# Autodesk Inventor assembly: 276-2181
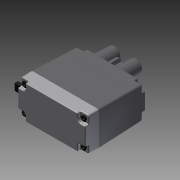
[picture p0: Inventor's stored thumbnail of the model, 180x180]
Saved by Autodesk Inventor 2013 (Build 170138000, 138)
## iProperties
Category: Motors
Company: Autodesk Inc.
Created: 2012-01-28
Part Number: 276-2181
Document SubType Name: Assembly
Designer: Autodesk Inc.
Catalog Web Link: http://www.vexrobotics.com/276-2181.html
Vendor: VEX
Author: Autodesk Inc.
## Documents named in this file (18)
- C:\Data Folder\VEX 2012\VEX KOP Uploads\2013\Imperial\Motion\2-Wire Motor 269.iam
- C:\Data Folder\VEX 2012\VEX KOP Uploads\2013\Imperial\Motion\Components\276-2181-002 Rev1.ipt
- C:\Data Folder\VEX 2012\VEX KOP Uploads\2013\Imperial\Motion\Components\276-2181-006 Rev1.ipt
- C:\Data Folder\VEX 2012\VEX KOP Uploads\2013\Imperial\Motion\Components\276-2181-011 Rev1.ipt
- C:\Data Folder\VEX 2012\VEX KOP Uploads\2013\Imperial\Motion\Components\276-2177-018 Rev1.ipt
- C:\Data Folder\VEX 2012\VEX KOP Uploads\2013\Imperial\Motion\Components\276-2181-004 Rev1.ipt
- C:\Data Folder\VEX 2012\VEX KOP Uploads\2013\Imperial\Motion\Components\276-2181-008 Rev1_276-2181-008g.ipt
- C:\Data Folder\VEX 2012\VEX KOP Uploads\2013\Imperial\Motion\Components\276-2181-007 Rev1.ipt
- C:\Data Folder\VEX 2012\VEX KOP Uploads\2013\Imperial\Motion\Components\276-2181-012 Rev1.ipt
- C:\Data Folder\VEX 2012\VEX KOP Uploads\2013\Imperial\Motion\Components\276-2181-003 Rev1.ipt
- C:\Data Folder\VEX 2012\VEX KOP Uploads\2013\Imperial\Motion\Components\276-2181-001 Rev1.ipt
- C:\Data Folder\VEX 2012\VEX KOP Uploads\2013\Imperial\Motion\Components\QFK-N30QAV-16068.ipt
- C:\Data Folder\VEX 2012\VEX KOP Uploads\2013\Imperial\Motion\Components\ANSI B18.6.3 - 0-80 UNF - 0.1875(14).ipt
- C:\Data Folder\VEX 2012\VEX KOP Uploads\2013\Imperial\Motion\Components\276-2181-010 Rev1.ipt
- C:\Data Folder\VEX 2012\VEX KOP Uploads\2013\Imperial\Motion\Components\276-2181-009 Rev1.ipt
- C:\Data Folder\VEX 2012\VEX KOP Uploads\2013\Imperial\Motion\Components\276-2181-005 Rev1.ipt
- C:\Data Folder\VEX 2012\VEX KOP Uploads\2013\Imperial\Motion\Components\276-2177-019 Rev1.ipt
- C:\Data Folder\VEX 2012\VEX KOP Uploads\2013\Imperial\Motion\Components\ANSI B18.6.3 - 0-80 UNF - 0.5(17).ipt
## Components (29 placed, 17 different names)
1. 276-2181-002 Rev1:1 — Insert:1, Insert:2, Mate:1, Mate:3, Insert:3, Mate:4, Flush:1, Mate:5, Mate:9, Mate:10, Mate:11, Mate:12, Mate:13, Mate:14, Angle:1, Insert:5, Mate:15, Insert:6, Insert:7, Mate:16, Insert:8, Flush:2, Flush:3, Flush:4
2. 276-2181-006 Rev1:1 — Insert:1, Mate:18
3. 276-2181-011 Rev1:1 — Insert:2, Insert:4
4. 276-2177-018 Rev1:1 — Mate:1, Mate:3
5. 276-2181-004 Rev1:1 — Insert:3
6. 276-2181-008 Rev1_276-2181-008g:1 — Insert:4, Insert:9
7. 276-2181-007 Rev1:1 — Mate:4, Flush:1, Mate:7, Mate:8
8. 276-2181-012 Rev1:1 — Mate:5, Angle:1, Mate:19
9. 276-2181-006 Rev1:2 — Mate:7, Mate:8, Mate:17
10. 276-2181-003 Rev1:1 — Mate:9, Mate:10, Mate:14, Insert:10, Insert:11, Insert:16, Insert:17, Insert:18, Insert:19
11. 276-2181-001 Rev1:1 — Mate:11, Mate:12, Mate:13, Insert:12, Insert:13, Insert:14, Insert:15
12. QFK-N30QAV-16068:1 — Insert:5, Mate:15, Mate:19
13. Cross Recessed Binding Head Machine Screw - Type I - Inch 0 - 80 - 3/16:1 — Insert:6
14. Cross Recessed Binding Head Machine Screw - Type I - Inch 0 - 80 - 3/16:2 — Insert:7
15. 276-2181-010 Rev1:1 — Mate:16, Flush:2
16. 276-2181-009 Rev1:1 — Mate:17, Flush:3
17. 276-2181-005 Rev1:1 — Insert:8
18. 276-2181-010 Rev1:2 — Mate:18, Flush:4
19. 276-2181-011 Rev1:2 — Insert:9
20. 276-2177-019 Rev1:1 — Insert:10
21. 276-2177-019 Rev1:2 — Insert:11
22. Cross Recessed Binding Head Machine Screw - Type II - Inch 0 - 80 - 1/2:1 — Insert:12
23. Cross Recessed Binding Head Machine Screw - Type II - Inch 0 - 80 - 1/2:2 — Insert:13
24. Cross Recessed Binding Head Machine Screw - Type II - Inch 0 - 80 - 1/2:4 — Insert:15
25. Cross Recessed Binding Head Machine Screw - Type II - Inch 0 - 80 - 1/2:3 — Insert:14
26. Cross Recessed Binding Head Machine Screw - Type II - Inch 0 - 80 - 1/2:5 — Insert:16
27. Cross Recessed Binding Head Machine Screw - Type II - Inch 0 - 80 - 1/2:6 — Insert:17
28. Cross Recessed Binding Head Machine Screw - Type II - Inch 0 - 80 - 1/2:7 — Insert:18
29. Cross Recessed Binding Head Machine Screw - Type II - Inch 0 - 80 - 1/2:8 — Insert:19
## Relationships (41: Insert 19, Mate 17, Flush 4, Angle 1)
- Insert:1: 276-2181-002 Rev1:1 ↔ 276-2181-006 Rev1:1
- Insert:2: 276-2181-002 Rev1:1 ↔ 276-2181-011 Rev1:1
- Mate:1: 276-2181-002 Rev1:1 ↔ 276-2177-018 Rev1:1
- Mate:3: 276-2181-002 Rev1:1 ↔ 276-2177-018 Rev1:1
- Insert:3: 276-2181-002 Rev1:1 ↔ 276-2181-004 Rev1:1
- Insert:4: 276-2181-011 Rev1:1 ↔ 276-2181-008 Rev1_276-2181-008g:1
- Mate:4: 276-2181-002 Rev1:1 ↔ 276-2181-007 Rev1:1
- Flush:1 (4.191 mm): 276-2181-002 Rev1:1 ↔ 276-2181-007 Rev1:1
- Mate:5: 276-2181-002 Rev1:1 ↔ 276-2181-012 Rev1:1
- Mate:7: 276-2181-007 Rev1:1 ↔ 276-2181-006 Rev1:2
- Mate:8: 276-2181-007 Rev1:1 ↔ 276-2181-006 Rev1:2
- Mate:9: 276-2181-002 Rev1:1 ↔ 276-2181-003 Rev1:1
- Mate:10: 276-2181-002 Rev1:1 ↔ 276-2181-003 Rev1:1
- Mate:11: 276-2181-002 Rev1:1 ↔ 276-2181-001 Rev1:1
- Mate:12: 276-2181-002 Rev1:1 ↔ 276-2181-001 Rev1:1
- Mate:13: 276-2181-002 Rev1:1 ↔ 276-2181-001 Rev1:1
- Mate:14: 276-2181-002 Rev1:1 ↔ 276-2181-003 Rev1:1
- Angle:1 (0 deg): 276-2181-002 Rev1:1 ↔ 276-2181-012 Rev1:1
- Insert:5: 276-2181-002 Rev1:1 ↔ QFK-N30QAV-16068:1
- Mate:15: 276-2181-002 Rev1:1 ↔ QFK-N30QAV-16068:1
- Insert:6: 276-2181-002 Rev1:1 ↔ Cross Recessed Binding Head Machine Screw - Type I - Inch 0 - 80 - 3/16:1
- Insert:7: 276-2181-002 Rev1:1 ↔ Cross Recessed Binding Head Machine Screw - Type I - Inch 0 - 80 - 3/16:2
- Mate:16: 276-2181-002 Rev1:1 ↔ 276-2181-010 Rev1:1
- Insert:8: 276-2181-002 Rev1:1 ↔ 276-2181-005 Rev1:1
- Flush:2 (8.1026 mm): 276-2181-002 Rev1:1 ↔ 276-2181-010 Rev1:1
- Mate:17: 276-2181-006 Rev1:2 ↔ 276-2181-009 Rev1:1
- Flush:3 (12.9032 mm): 276-2181-002 Rev1:1 ↔ 276-2181-009 Rev1:1
- Mate:18: 276-2181-006 Rev1:1 ↔ 276-2181-010 Rev1:2
- Flush:4 (13.1064 mm): 276-2181-002 Rev1:1 ↔ 276-2181-010 Rev1:2
- Mate:19: 276-2181-012 Rev1:1 ↔ QFK-N30QAV-16068:1
- Insert:9: 276-2181-008 Rev1_276-2181-008g:1 ↔ 276-2181-011 Rev1:2
- Insert:10 (-0.6096 mm): 276-2181-003 Rev1:1 ↔ 276-2177-019 Rev1:1
- Insert:11 (-0.6096 mm): 276-2181-003 Rev1:1 ↔ 276-2177-019 Rev1:2
- Insert:12: 276-2181-001 Rev1:1 ↔ Cross Recessed Binding Head Machine Screw - Type II - Inch 0 - 80 - 1/2:1
- Insert:13: 276-2181-001 Rev1:1 ↔ Cross Recessed Binding Head Machine Screw - Type II - Inch 0 - 80 - 1/2:2
- Insert:14: 276-2181-001 Rev1:1 ↔ Cross Recessed Binding Head Machine Screw - Type II - Inch 0 - 80 - 1/2:3
- Insert:15: 276-2181-001 Rev1:1 ↔ Cross Recessed Binding Head Machine Screw - Type II - Inch 0 - 80 - 1/2:4
- Insert:16: 276-2181-003 Rev1:1 ↔ Cross Recessed Binding Head Machine Screw - Type II - Inch 0 - 80 - 1/2:5
- Insert:17: 276-2181-003 Rev1:1 ↔ Cross Recessed Binding Head Machine Screw - Type II - Inch 0 - 80 - 1/2:6
- Insert:18: 276-2181-003 Rev1:1 ↔ Cross Recessed Binding Head Machine Screw - Type II - Inch 0 - 80 - 1/2:7
- Insert:19: 276-2181-003 Rev1:1 ↔ Cross Recessed Binding Head Machine Screw - Type II - Inch 0 - 80 - 1/2:8
